# Autodesk Inventor assembly: gearhub_mirrored
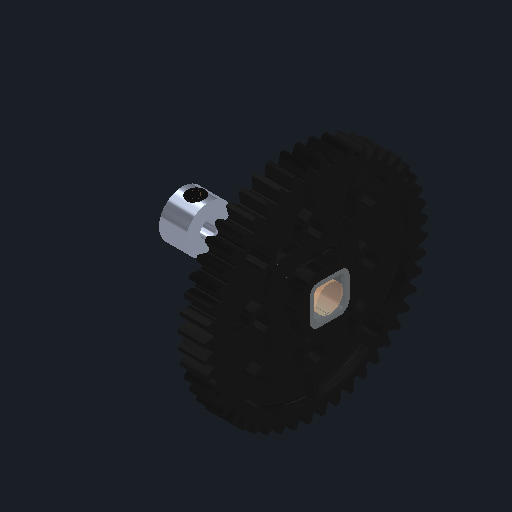
[picture p0: Inventor's stored thumbnail of the model, 512x512]
Saved by Autodesk Inventor 2025 (Build 290162000, 162)
## iProperties
Created: 2024-06-25
Part Number: gearhub_mirrored
Document SubType Name: Assembly
Designer: Averey Ku
Author: Audrey
## Documents named in this file (3)
- D:\vex_robotics_high_stakes\hardware\cad\EARLY_SEASON\chassis\mirrored_parts\gearhub_mirrored.iam
- D:\vex_robotics_high_stakes\hardware\cad\EARLY_SEASON\chassis\mirrored_parts\Shaft Collar Set Screw_mirrored.ipt
- D:\vex_robotics_high_stakes\hardware\cad\EARLY_SEASON\chassis\mirrored_parts\Half Cut HS 48T Gear, No Insert_mirrored.ipt
## Components (3 placed, 2 different names)
1. Shaft Collar Set Screw_mirrored:1 — Insert:1
2. Shaft Collar Set Screw_mirrored:2 — Insert:1, Insert:2
3. Half Cut HS 48T Gear, No Insert_mirrored:1 — Insert:2
## Relationships (2: Insert 2)
- Insert:1 (9.525 mm): Shaft Collar Set Screw_mirrored:1 ↔ Shaft Collar Set Screw_mirrored:2
- Insert:2: Shaft Collar Set Screw_mirrored:2 ↔ Half Cut HS 48T Gear, No Insert_mirrored:1
